# Autodesk Inventor assembly: top
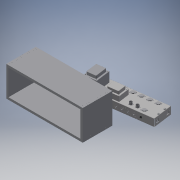
[picture p0: Inventor's stored thumbnail of the model, 180x180]
Saved by Autodesk Inventor 2016 (Build 200138000, 138)
## iProperties
Created: 2015-10-24
Part Number: top
Document SubType Name: Assembly
Designer: jeremyhale
Author: jeremyhale
## Documents named in this file (4)
- \\psf\Home\Documents\Poorhouse\git\p0001\top.iam
- \\psf\Home\Documents\Poorhouse\git\p0001\cabinet.iam
- \\psf\Home\Documents\Poorhouse\git\p0001\chassis.iam
- chassis.iam
## Components (2 placed, 2 different names)
1. cabinet:1 [sub-assembly] — Mate:1
2. chassis:1 [sub-assembly] — Mate:1
## Relationships (1: Mate 1)
- Mate:1: cabinet:1 ↔ chassis:1
